# Autodesk Inventor assembly: Left-Arm-Base
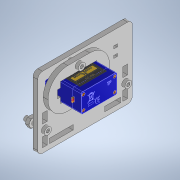
[picture p0: Inventor's stored thumbnail of the model, 180x180]
Saved by Autodesk Inventor 2022 (Build 260153000, 153)
## iProperties
Created: 2020-02-05
Part Number: Left-Arm-Base
Document SubType Name: Assembly
Designer: joshn
Author: joshn
Revision Number: NONE
## Documents named in this file (10)
- D:\Joshwin Emmanuel\Fab_accad\git_hub\Fab_Work\arm\step\part\Left-Arm-Base.iam
- D:\Joshwin Emmanuel\Fab_accad\git_hub\Fab_Work\arm\step\part\NONE_4.ipt
- D:\Joshwin Emmanuel\Fab_accad\git_hub\Fab_Work\arm\step\part\Left Arm Servo Plate.ipt
- D:\Joshwin Emmanuel\Fab_accad\git_hub\Fab_Work\arm\step\part\Schraube _ Zylinder - M3,0 x 8,0_3.ipt
- D:\Joshwin Emmanuel\Fab_accad\git_hub\Fab_Work\arm\step\part\Schraube _ Zylinder - M3,0 x 8,0_4.ipt
- D:\Joshwin Emmanuel\Fab_accad\git_hub\Fab_Work\arm\step\part\Zyl-Imbus M3x12_2.ipt
- D:\Joshwin Emmanuel\Fab_accad\git_hub\Fab_Work\arm\step\part\Mutter _  - M3,0 x 57,785_3.ipt
- D:\Joshwin Emmanuel\Fab_accad\git_hub\Fab_Work\arm\step\part\Mutter _  - M3,0 x 57,785_4.ipt
- D:\Joshwin Emmanuel\Fab_accad\git_hub\Fab_Work\arm\step\part\Zyl-Imbus M3x12_3.ipt
- D:\Joshwin Emmanuel\Fab_accad\git_hub\Fab_Work\arm\step\part\SG90 - Micro Servo 9g - Tower Pro.1.ipt
## Components (9 placed, 6 different names)
1. Servo Retainer — Mate:1
2. Left Arm Servo Plate — Mate:2, Mate:3
3. SG90 - Micro Servo 9g - Tower Pro.1:1 — Mate:1, Mate:2, Mate:3
4. Schraube : Zylinder - M3,0 x 8,0
5. Schraube : Zylinder - M3,0 x 8,0:1
6. Zyl-Imbus M3x12
7. Mutter :  - M3,0 x 57,785
8. Mutter :  - M3,0 x 57,785:1
9. Zyl-Imbus M3x12:1
## Relationships (3: Mate 3)
- Mate:1: Servo Retainer ↔ SG90 - Micro Servo 9g - Tower Pro.1:1
- Mate:2: Left Arm Servo Plate ↔ SG90 - Micro Servo 9g - Tower Pro.1:1
- Mate:3: Left Arm Servo Plate ↔ SG90 - Micro Servo 9g - Tower Pro.1:1
